# Autodesk Inventor assembly: test
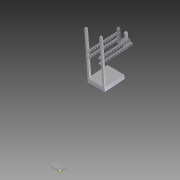
[picture p0: Inventor's stored thumbnail of the model, 180x180]
Saved by Autodesk Inventor 2015 (Build 190159000, 159)
## iProperties
Created: 2015-01-15
Part Number: test
Document SubType Name: Assembly
Designer: Tucker
Author: Tucker
## Documents named in this file (7)
- C:\Users\Tucker\Documents\GitHub\frc2015\CAD\test.iam
- C:\Users\Tucker\Documents\GitHub\frc2015\CAD\chasse.ipt
- C:\Users\Tucker\Documents\GitHub\frc2015\CAD\pole.ipt
- C:\Users\Tucker\Documents\GitHub\frc2015\CAD\box_forklift.ipt
- C:\Users\Tucker\Documents\GitHub\frc2015\CAD\axle_word_used_loosely.ipt
- C:\Users\Tucker\Documents\GitHub\frc2015\CAD\gripper_mc_dipper.ipt
- C:\Users\Tucker\Documents\GitHub\frc2015\CAD\pole_2.ipt
## Components (19 placed, 6 different names)
1. chasse:1 — Mate:1, Flush:1, Flush:2, Mate:2, Flush:3, Flush:4
2. pole:1 — Mate:1, Flush:1, Flush:2, Mate:3, Rotation:1, Mate:4, Mate:6, Mate:7, Flush:6
3. pole:2 — Mate:2, Flush:3, Flush:4, Mate:5, Mate:8, Flush:5, Flush:7
4. box_forklift:1
5. axle_word_used_loosely:1 — Mate:3, Rotation:1, Mate:4, Flush:6, Mate:21, Mate:22
6. axle_word_used_loosely:2 — Mate:6, Mate:7, Mate:23, Mate:24
7. axle_word_used_loosely:3 — Mate:5, Flush:7, Mate:25, Mate:26
8. axle_word_used_loosely:4 — Mate:8, Flush:5, Mate:27, Mate:28
9. gripper_mc_dipper:2 — Flush:10, Mate:31, Mate:32, Mate:33, Flush:11, Flush:12
10. axle_word_used_loosely:5 — Mate:29, Flush:8, Flush:10, Mate:31
11. pole_2:1 — Mate:21, Mate:22, Mate:29, Flush:8
12. pole_2:2 — Mate:23, Mate:24, Mate:30, Flush:9
13. pole_2:3 — Mate:25, Mate:26, Mate:34, Flush:13
14. pole_2:4 — Mate:27, Mate:28, Mate:35, Flush:14
15. axle_word_used_loosely:6 — Mate:30, Flush:9, Mate:32
16. box_forklift:2 — Mate:33, Flush:11, Flush:12, Mate:38
17. axle_word_used_loosely:7 — Mate:35, Flush:14, Mate:37, Flush:16
18. axle_word_used_loosely:8 — Mate:34, Flush:13, Mate:36, Flush:15
19. gripper_mc_dipper:3 — Mate:36, Mate:37, Flush:15, Flush:16, Mate:38
## Relationships (43: Mate 26, Flush 16, RelateRotation 1)
- Mate:1: chasse:1 ↔ pole:1
- Flush:1: chasse:1 ↔ pole:1
- Flush:2: chasse:1 ↔ pole:1
- Mate:2: chasse:1 ↔ pole:2
- Flush:3: chasse:1 ↔ pole:2
- Flush:4: chasse:1 ↔ pole:2
- Mate:3: pole:1 ↔ axle_word_used_loosely:1
- Rotation:1 [RelateRotation] (1 ul): pole:1 ↔ axle_word_used_loosely:1
- Mate:4: pole:1 ↔ axle_word_used_loosely:1
- Mate:5: pole:2 ↔ axle_word_used_loosely:3
- Mate:6: pole:1 ↔ axle_word_used_loosely:2
- Mate:7: pole:1 ↔ axle_word_used_loosely:2
- Mate:8: pole:2 ↔ axle_word_used_loosely:4
- Flush:5: pole:2 ↔ axle_word_used_loosely:4
- Flush:6: pole:1 ↔ axle_word_used_loosely:1
- Flush:7: pole:2 ↔ axle_word_used_loosely:3
- Mate:21: axle_word_used_loosely:1 ↔ pole_2:1
- Mate:22: axle_word_used_loosely:1 ↔ pole_2:1
- Mate:23: axle_word_used_loosely:2 ↔ pole_2:2
- Mate:24: axle_word_used_loosely:2 ↔ pole_2:2
- Mate:25: axle_word_used_loosely:3 ↔ pole_2:3
- Mate:26: axle_word_used_loosely:3 ↔ pole_2:3
- Mate:27: axle_word_used_loosely:4 ↔ pole_2:4
- Mate:28: axle_word_used_loosely:4 ↔ pole_2:4
- Mate:29: axle_word_used_loosely:5 ↔ pole_2:1
- Flush:8: axle_word_used_loosely:5 ↔ pole_2:1
- Mate:30: pole_2:2 ↔ axle_word_used_loosely:6
- Flush:9: pole_2:2 ↔ axle_word_used_loosely:6
- Flush:10: gripper_mc_dipper:2 ↔ axle_word_used_loosely:5
- Mate:31: gripper_mc_dipper:2 ↔ axle_word_used_loosely:5
- Mate:32: gripper_mc_dipper:2 ↔ axle_word_used_loosely:6
- Mate:33: gripper_mc_dipper:2 ↔ box_forklift:2
- Flush:11: gripper_mc_dipper:2 ↔ box_forklift:2
- Flush:12: gripper_mc_dipper:2 ↔ box_forklift:2
- Mate:34: pole_2:3 ↔ axle_word_used_loosely:8
- Flush:13: pole_2:3 ↔ axle_word_used_loosely:8
- Mate:35: pole_2:4 ↔ axle_word_used_loosely:7
- Flush:14: pole_2:4 ↔ axle_word_used_loosely:7
- Mate:36: axle_word_used_loosely:8 ↔ gripper_mc_dipper:3
- Mate:37: axle_word_used_loosely:7 ↔ gripper_mc_dipper:3
- Flush:15: axle_word_used_loosely:8 ↔ gripper_mc_dipper:3
- Flush:16: axle_word_used_loosely:7 ↔ gripper_mc_dipper:3
- Mate:38: box_forklift:2 ↔ gripper_mc_dipper:3
